# Autodesk Inventor assembly: X_CarriageL_V2_0
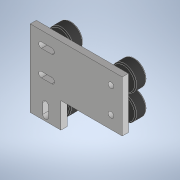
[picture p0: Inventor's stored thumbnail of the model, 180x180]
Saved by Autodesk Inventor 2021 (Build 250183000, 183)
## iProperties
Created: 2021-06-13
Part Number: X_CarriageL_V2_0
Document SubType Name: Assembly
Designer: Jorian Brusind
Author: Jorian Brusind
## Documents named in this file (3)
- C:\Users\Jorian Brusind\Documents\GitHub\PersonalProjects\HyperRail\Inventor Files\X_CarriageL_V2_0.iam
- C:\Users\Jorian Brusind\Documents\GitHub\PersonalProjects\HyperRail\Inventor Files\X_Carriage_Plate.ipt
- C:\Users\Jorian Brusind\Documents\GitHub\PersonalProjects\HyperRail\Inventor Files\11mm_BearingWheel.ipt
## Components (6 placed, 2 different names)
1. X_Carriage_Plate:1 — Mate:1, Mate:2, Mate:3, Mate:5, Mate:7, Mate:8, Mate:9, Mate:10
2. 11mm_BearingWheel:1 — Mate:1, Mate:6, Flush:2
3. 11mm_BearingWheel:2 — Mate:5, Mate:6, Flush:1
4. 11mm_BearingWheel:3 — Mate:3, Mate:4, Flush:1, Flush:3
5. 11mm_BearingWheel:4 — Mate:2, Mate:4, Flush:2, Flush:3, Mate:7
6. 11mm_BearingWheel:5 — Mate:8, Mate:9, Mate:10
## Relationships (13: Mate 10, Flush 3)
- Mate:1: X_Carriage_Plate:1 ↔ 11mm_BearingWheel:1
- Mate:2: X_Carriage_Plate:1 ↔ 11mm_BearingWheel:4
- Mate:3 (2.75 mm): X_Carriage_Plate:1 ↔ 11mm_BearingWheel:3
- Mate:4 (62 mm): 11mm_BearingWheel:3 ↔ 11mm_BearingWheel:4
- Mate:5 (2.75 mm): X_Carriage_Plate:1 ↔ 11mm_BearingWheel:2
- Mate:6 (62 mm): 11mm_BearingWheel:1 ↔ 11mm_BearingWheel:2
- Flush:1: 11mm_BearingWheel:2 ↔ 11mm_BearingWheel:3
- Flush:2: 11mm_BearingWheel:1 ↔ 11mm_BearingWheel:4
- Flush:3: 11mm_BearingWheel:3 ↔ 11mm_BearingWheel:4
- Mate:7 (6 mm): X_Carriage_Plate:1 ↔ 11mm_BearingWheel:4
- Mate:8 (2.75 mm): X_Carriage_Plate:1 ↔ 11mm_BearingWheel:5
- Mate:9 (-10 mm): X_Carriage_Plate:1 ↔ 11mm_BearingWheel:5
- Mate:10 (6 mm): X_Carriage_Plate:1 ↔ 11mm_BearingWheel:5
